# Autodesk Inventor assembly: draftFullAssembly
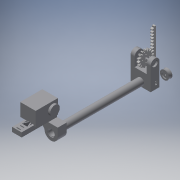
[picture p0: Inventor's stored thumbnail of the model, 180x180]
Saved by Autodesk Inventor 2017 (Build 210142000, 142)
## iProperties
Created: 2018-10-18
Part Number: draftFullAssembly
Document SubType Name: Assembly
Designer: Tom
Author: Tom
## Documents named in this file (5)
- C:\Users\Tom\Google Drive\UQ\UNI_WORK\METR4202\Problem Sets\PS3\CAD\draftFullAssembly.iam
- C:\Users\Tom\Google Drive\UQ\UNI_WORK\METR4202\Problem Sets\PS3\CAD\HectorsArm.ipt
- C:\Users\Tom\Google Drive\UQ\UNI_WORK\METR4202\Problem Sets\PS3\CAD\draftEndEffectorV2.iam
- C:\Users\Tom\Google Drive\UQ\UNI_WORK\METR4202\Problem Sets\PS3\CAD\HousingV4.ipt
- C:\Users\Tom\Google Drive\UQ\UNI_WORK\METR4202\Problem Sets\PS3\CAD\motor.ipt
## Components (4 placed, 4 different names)
1. HectorsArm:1 — Mate:1, Mate:2, Mate:3
2. draftEndEffectorV2:1 [sub-assembly] — Mate:2, Mate:3
3. HousingV4:1 — Mate:1, Mate:4, Mate:5
4. motor:1 — Mate:4, Mate:5
## Relationships (5: Mate 5)
- Mate:1: HectorsArm:1 ↔ HousingV4:1
- Mate:2: HectorsArm:1 ↔ draftEndEffectorV2:1
- Mate:3: HectorsArm:1 ↔ draftEndEffectorV2:1
- Mate:4: HousingV4:1 ↔ motor:1
- Mate:5: HousingV4:1 ↔ motor:1
